# Autodesk Inventor assembly: FalconMod
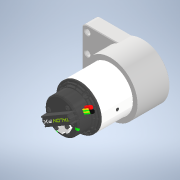
[picture p0: Inventor's stored thumbnail of the model, 180x180]
Saved by Autodesk Inventor 2020 (Build 240168000, 168)
## iProperties
Created: 2020-02-18
Part Number: FalconMod
Document SubType Name: Assembly
Designer: srini
Author: srini
## Documents named in this file (6)
- C:\Users\srini\Documents\FRC\2020\FalconMod.iam
- C:\Users\srini\Documents\FRC\2020\BearingStandoff2Falcon.ipt
- C:\Users\srini\Documents\FRC\2020\Shooter\Falcon_500_Powered_by_Talon_FX_217-6515.iam
- C:\Users\srini\Documents\FRC\2020\Shooter\217-5839-006 Rev4.ipt
- C:\Users\srini\Documents\FRC\2020\Shooter\VP_Press_On_Motor_Coupler_Falcon_Motor_217-6789.ipt
- C:\Users\srini\Documents\FRC\2020\IntakeShooter\13_75mm_1_2_ThunderHex_ID_x_1_125_OD_x_0_313_WD_Flanged_Bearing_217-4006_MIR1.ipt
## Components (5 placed, 5 different names)
1. BearingStandoff2Falcon:1 — Insert:1, Insert:4
2. Falcon_500_Powered_by_Talon_FX_217-6515:1 [sub-assembly] — Insert:1, Insert:2
3. 217-5839-006 Rev4:1 — Insert:3
4. VP_Press_On_Motor_Coupler_Falcon_Motor_217-6789:1 — Insert:2, Insert:3
5. 13_75mm_1_2_ThunderHex_ID_x_1_125_OD_x_0_313_WD_Flanged_Bearing_217-4006_MIR1:1 — Insert:4
## Relationships (4: Insert 4)
- Insert:1 (19.05 mm): BearingStandoff2Falcon:1 ↔ Falcon_500_Powered_by_Talon_FX_217-6515:1
- Insert:2: Falcon_500_Powered_by_Talon_FX_217-6515:1 ↔ VP_Press_On_Motor_Coupler_Falcon_Motor_217-6789:1
- Insert:3: 217-5839-006 Rev4:1 ↔ VP_Press_On_Motor_Coupler_Falcon_Motor_217-6789:1
- Insert:4: BearingStandoff2Falcon:1 ↔ 13_75mm_1_2_ThunderHex_ID_x_1_125_OD_x_0_313_WD_Flanged_Bearing_217-4006_MIR1:1
